# Autodesk Inventor assembly: A90T_7
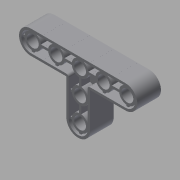
[picture p0: Inventor's stored thumbnail of the model, 180x180]
Saved by Autodesk Inventor 2019.3 (Build 233278000, 278)
## iProperties
Created: 2019-02-01
Part Number: A90T_7
Document SubType Name: Assembly
Designer: Varga Daniel
Vertical_hole_count: 3,000 ul
Horizontal_hole_count_right: 3,000 ul
Horizontal_hole_count_left: 3,000 ul
Author: Varga Daniel
## Documents named in this file (5)
- C:\!_Dani\!_cloud\OneDrive\!_munka\Revolution\RevvyDemoKit\Structural parts\Beams\Angled Beams\T shape beams\A90T_7.iam
- C:\!_Dani\!_cloud\OneDrive\!_munka\Revolution\RevvyDemoKit\Structural parts\Beams\beam_single_inner_part.ipt
- C:\!_Dani\!_cloud\OneDrive\!_munka\Revolution\RevvyDemoKit\Structural parts\Beams\beam_single_end_part.ipt
- C:\!_Dani\!_cloud\OneDrive\!_munka\Revolution\RevvyDemoKit\Structural parts\Beams\Angled Beams\T beam base.ipt
- C:\!_Dani\!_cloud\OneDrive\!_munka\Revolution\RevvyDemoKit\Structural parts\Beams\Angled Beams\T shape beams.iam
## Components (7 placed, 3 different names)
1. beam_single_end_part:1 — Flush:1, Flush:2, Mate:1
2. T beam base:1 — Flush:1, Flush:2, Mate:1, Flush:3, Flush:4, Mate:2, Flush:5, Flush:6, Mate:3, Flush:7, Flush:8, Mate:4, Flush:9, Flush:10, Mate:5, Flush:11, Flush:12, Mate:6
3. beam_single_end_part:2 — Flush:3, Flush:4, Mate:2
4. beam_single_end_part:3 — Flush:5, Flush:6, Mate:3
5. beam_single_inner_part:3 — Flush:9, Flush:10, Mate:5
6. beam_single_inner_part:2 — Flush:7, Flush:8, Mate:4
7. beam_single_inner_part:1 — Flush:11, Flush:12, Mate:6
## Component patterns: (1 elements, first: beam_single_inner_part:3), (1 elements, first: beam_single_inner_part:2), (1 elements, first: beam_single_inner_part:1)
## Relationships (18: Flush 12, Mate 6)
- Flush:1: beam_single_end_part:1 ↔ T beam base:1
- Flush:2: beam_single_end_part:1 ↔ T beam base:1
- Mate:1 (10 mm): beam_single_end_part:1 ↔ T beam base:1
- Flush:3: T beam base:1 ↔ beam_single_end_part:2
- Flush:4: T beam base:1 ↔ beam_single_end_part:2
- Mate:2 (10 mm): T beam base:1 ↔ beam_single_end_part:2
- Flush:5: T beam base:1 ↔ beam_single_end_part:3
- Flush:6: T beam base:1 ↔ beam_single_end_part:3
- Mate:3 (10 mm): T beam base:1 ↔ beam_single_end_part:3
- Flush:7: T beam base:1 ↔ beam_single_inner_part:2
- Flush:8: T beam base:1 ↔ beam_single_inner_part:2
- Mate:4: T beam base:1 ↔ beam_single_inner_part:2
- Flush:9: T beam base:1 ↔ beam_single_inner_part:3
- Flush:10: T beam base:1 ↔ beam_single_inner_part:3
- Mate:5: T beam base:1 ↔ beam_single_inner_part:3
- Flush:11: T beam base:1 ↔ beam_single_inner_part:1
- Flush:12: T beam base:1 ↔ beam_single_inner_part:1
- Mate:6: T beam base:1 ↔ beam_single_inner_part:1
